# Autodesk Inventor assembly: omni_wheel
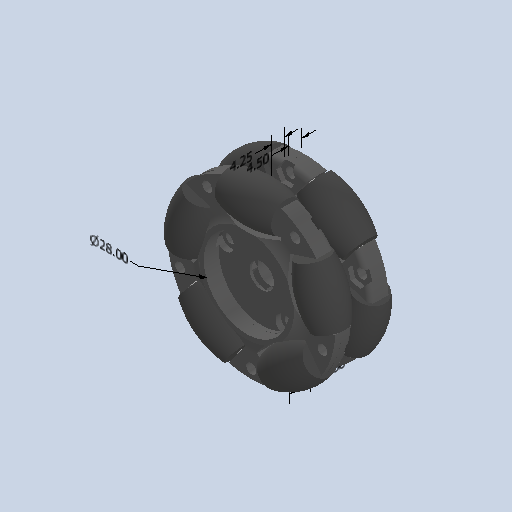
[picture p0: Inventor's stored thumbnail of the model, 512x512]
Saved by Autodesk Inventor 2024.1 (Build 281209000, 209)
## iProperties
Created: 2024-12-18
Part Number: omni_wheel
Document SubType Name: Assembly
Designer: hibik
Author: hibik
## Documents named in this file (6)
- C:\Users\hibik\Documents\Robomech\RESCUE\ORCA\hard\omni_wheel\omni_wheel.iam
- C:\Users\hibik\Documents\Robomech\RESCUE\ORCA\hard\omni_wheel\wheel_body_back_inside.ipt
- C:\Users\hibik\Documents\Robomech\RESCUE\ORCA\hard\omni_wheel\wheel_body_front_inside.ipt
- C:\Users\hibik\Documents\Robomech\RESCUE\ORCA\hard\omni_wheel\wheel_body_back_outside.ipt
- C:\Users\hibik\Documents\Robomech\RESCUE\ORCA\hard\omni_wheel\wheel_body_front_outside.ipt
- C:\Users\hibik\Documents\Robomech\RESCUE\ORCA\hard\omni_wheel\roller.ipt
## Components (14 placed, 5 different names)
1. wheel_body_front_outside:1 — 挿入:5, 挿入:6, フラッシュ:1
2. wheel_body_back_inside:1 — 挿入:1, 挿入:2, 挿入:4, フラッシュ:1, 挿入:8, 正接:3, 正接:4, メイト:2
3. wheel_body_back_outside:1 — 挿入:4, 挿入:5, 挿入:6, 挿入:8, 正接:1, 正接:2, メイト:1
4. wheel_body_front_inside:1 — 挿入:1, 挿入:2
5. roller:1 — 正接:1, 正接:2, メイト:1
6. roller:3
7. roller:4
8. roller:5
9. roller:6
10. roller:2 — 正接:3, 正接:4, メイト:2
11. roller:7
12. roller:8
13. roller:9
14. roller:10
## Component patterns: (5 elements, first: roller:1), (5 elements, first: roller:2)
## Relationships (13: Insert 6, Tangent 4, Mate 2, Flush 1)
- 挿入:1 [Insert]: wheel_body_back_inside:1 ↔ wheel_body_front_inside:1
- 挿入:2 [Insert]: wheel_body_back_inside:1 ↔ wheel_body_front_inside:1
- 挿入:4 [Insert]: wheel_body_back_inside:1 ↔ wheel_body_back_outside:1
- 挿入:5 [Insert]: wheel_body_front_outside:1 ↔ wheel_body_back_outside:1
- 挿入:6 [Insert]: wheel_body_front_outside:1 ↔ wheel_body_back_outside:1
- フラッシュ:1 [Flush]: wheel_body_front_outside:1 ↔ wheel_body_back_inside:1
- 挿入:8 [Insert]: wheel_body_back_inside:1 ↔ wheel_body_back_outside:1
- 正接:1 [Tangent]: wheel_body_back_outside:1 ↔ roller:1
- 正接:2 [Tangent]: wheel_body_back_outside:1 ↔ roller:1
- メイト:1 [Mate] (0.5 mm): wheel_body_back_outside:1 ↔ roller:1
- 正接:3 [Tangent]: wheel_body_back_inside:1 ↔ roller:2
- 正接:4 [Tangent]: wheel_body_back_inside:1 ↔ roller:2
- メイト:2 [Mate] (0.5 mm): wheel_body_back_inside:1 ↔ roller:2
